# Autodesk Inventor assembly: Puzzle Cube
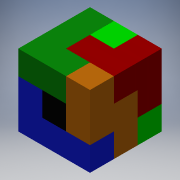
[picture p0: Inventor's stored thumbnail of the model, 180x180]
Saved by Autodesk Inventor 2018 (Build 220112000, 112)
## iProperties
Created: 2019-12-10
Part Number: Puzzle Cube
Document SubType Name: Assembly
Designer: zasi5b1
Author: zasi5b1
## Documents named in this file (7)
- I:\CAD\Inventor Creations\Cube\Puzzle Cube.iam
- I:\CAD\Inventor Creations\Cube\Blue Cube Part.ipt
- I:\CAD\Inventor Creations\Cube\Black Cube Part.ipt
- I:\CAD\Inventor Creations\Cube\Orange Cube Part.ipt
- I:\CAD\Inventor Creations\Cube\Green Cube Part.ipt
- I:\CAD\Inventor Creations\Cube\Red Cube Part.ipt
- I:\CAD\Inventor Creations\Cube\Dark Green Cube Part.ipt
## Components (6 placed, 6 different names)
1. Blue Cube Part:1 — Flush:1, Flush:2, Flush:3, Flush:4, Flush:5, Flush:6, Mate:1, Flush:8
2. Black Cube Part:1 — Flush:1, Flush:2, Flush:3
3. Orange Cube Part:1 — Flush:4, Flush:5, Flush:6, Flush:7, Mate:3
4. Green Cube Part:1 — Mate:1, Flush:7, Flush:8, Flush:10, Mate:2, Flush:11, Flush:12, Mate:4
5. Red Cube Part:1 — Flush:10, Mate:2, Flush:11
6. Dark Green Cube Part:1 — Mate:3, Flush:12, Mate:4
## Relationships (15: Flush 11, Mate 4)
- Flush:1: Blue Cube Part:1 ↔ Black Cube Part:1
- Flush:2: Blue Cube Part:1 ↔ Black Cube Part:1
- Flush:3: Blue Cube Part:1 ↔ Black Cube Part:1
- Flush:4: Blue Cube Part:1 ↔ Orange Cube Part:1
- Flush:5: Blue Cube Part:1 ↔ Orange Cube Part:1
- Flush:6: Blue Cube Part:1 ↔ Orange Cube Part:1
- Mate:1: Blue Cube Part:1 ↔ Green Cube Part:1
- Flush:7: Orange Cube Part:1 ↔ Green Cube Part:1
- Flush:8: Blue Cube Part:1 ↔ Green Cube Part:1
- Flush:10: Green Cube Part:1 ↔ Red Cube Part:1
- Mate:2: Green Cube Part:1 ↔ Red Cube Part:1
- Flush:11: Green Cube Part:1 ↔ Red Cube Part:1
- Mate:3: Orange Cube Part:1 ↔ Dark Green Cube Part:1
- Flush:12: Green Cube Part:1 ↔ Dark Green Cube Part:1
- Mate:4: Green Cube Part:1 ↔ Dark Green Cube Part:1
